# Autodesk Inventor assembly: ASY ДМФ 01 50 Кассета
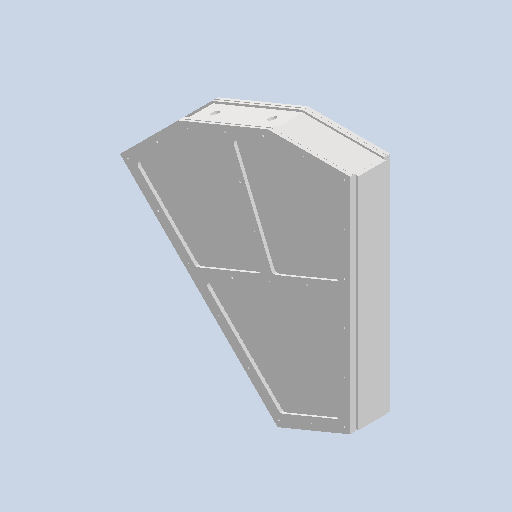
[picture p0: Inventor's stored thumbnail of the model, 512x512]
Saved by Autodesk Inventor 2024.2 (Build 282272000, 272)
## iProperties
Created: 2024-05-05
Part Number: ASY ДМФ 01 50 Кассета
Document SubType Name: Assembly
Designer: pokla
Author: pokla
## Documents named in this file (15)
- C:\Users\pokla\Documents\Inventor\ДФО\ДМФ\DMF-Disk-Micro-Filter-main 16.05.24 12-45\DMF-Disk-Micro-Filter-main\ASY ДМФ 01 50 Кассета.iam
- C:\Users\pokla\Documents\Inventor\ДФО\ДМФ\DMF-Disk-Micro-Filter-main 16.05.24 12-45\DMF-Disk-Micro-Filter-main\ДМФ 01 51 Внешняя рамка.ipt
- ДМС 201 Внешняя рамка.ipt
- C:\Users\pokla\Documents\Inventor\ДФО\ДМФ\DMF-Disk-Micro-Filter-main 16.05.24 12-45\DMF-Disk-Micro-Filter-main\ДМФ 01 52 Верхний лист.ipt
- C:\Users\pokla\Documents\Inventor\ДФО\ДМФ\DMF-Disk-Micro-Filter-main 16.05.24 12-45\DMF-Disk-Micro-Filter-main\ДМФ 01 53 Боковая часть.ipt
- C:\Users\pokla\Documents\Inventor\ДФО\ДМФ\DMF-Disk-Micro-Filter-main 16.05.24 12-45\DMF-Disk-Micro-Filter-main\ДМФ 01 54 Нижний лист.ipt
- C:\Users\pokla\Documents\Inventor\ДФО\ДМФ\DMF-Disk-Micro-Filter-main 16.05.24 12-45\DMF-Disk-Micro-Filter-main\ДМФ 01 55 Усилитель кассеты.ipt
- C:\Users\pokla\Documents\Inventor\ДФО\ДМФ\DMF-Disk-Micro-Filter-main 16.05.24 12-45\DMF-Disk-Micro-Filter-main\ДМФ 01 56 Крепление сетки к кассете.ipt
- ДМС 206 Крепление сетки к кассете.ipt
- C:\Users\pokla\Documents\Inventor\ДФО\ДМФ\DMF-Disk-Micro-Filter-main 16.05.24 12-45\DMF-Disk-Micro-Filter-main\ДМФ 01 57 Сетка кассеты.ipt
- ДМС 207 Сетка кассеты.ipt
- C:\Users\pokla\Documents\Inventor\ДФО\ДМФ\DMF-Disk-Micro-Filter-main 16.05.24 12-45\DMF-Disk-Micro-Filter-main\ДМФ 01 51 Внешние рамки_MIR1.ipt
- C:\Users\pokla\Documents\Inventor\ДФО\ДМФ\DMF-Disk-Micro-Filter-main 16.05.24 12-45\DMF-Disk-Micro-Filter-main\ДМФ 01 56 Крепление сетки к кассете_MIR1.ipt
- C:\Users\pokla\Documents\Inventor\ДФО\ДМФ\DMF-Disk-Micro-Filter-main 16.05.24 12-45\DMF-Disk-Micro-Filter-main\ДМФ 01 57 Сетка кассеты_MIR1.ipt
- C:\Users\pokla\Documents\Inventor\ДФО\ДМФ\DMF-Disk-Micro-Filter-main 16.05.24 12-45\DMF-Disk-Micro-Filter-main\ДМФ 01 58 Фиксатор расстояния кассет.ipt
## Components (12 placed, 11 different names)
1. ДМС 201 Внешняя рамка:1
2. ДМФ 01 52 Верхний лист:1
3. ДМФ 01 53 Боковая часть:1
4. ДМФ 01 54 Нижний лист:1
5. ДМФ 01 55 Усилитель кассеты:1
6. ДМС 206 Крепление сетки к кассете:1
7. ДМС 207 Сетка кассеты:1
8. ДМФ 01 53 Боковая часть:2
9. ДМФ 01 51 Внешние рамки_MIR1:1
10. ДМФ 01 56 Крепление сетки к кассете_MIR1:1
11. ДМФ 01 57 Сетка кассеты_MIR1:1
12. ДМФ 01 58 Фиксатор расстояния кассет:1
## Relationships (12: WeldJoint 8, RevoluteJoint 2, Mate 2)
- [WeldJoint]: ДМС 201 Внешняя рамка:1 ↔ ДМС 207 Сетка кассеты:1
- [WeldJoint]: ДМС 201 Внешняя рамка:1 ↔ ДМФ 01 52 Верхний лист:1
- [RevoluteJoint]: ДМС 201 Внешняя рамка:1 ↔ ДМФ 01 53 Боковая часть:1
- [Mate]: ДМС 201 Внешняя рамка:1 ↔ ДМФ 01 53 Боковая часть:1
- [WeldJoint] (0.5 mm): ДМС 201 Внешняя рамка:1 ↔ ДМС 206 Крепление сетки к кассете:1
- [RevoluteJoint]: ДМС 201 Внешняя рамка:1 ↔ ДМФ 01 53 Боковая часть:2
- [Mate]: ДМС 201 Внешняя рамка:1 ↔ ДМФ 01 53 Боковая часть:2
- [WeldJoint]: ДМС 201 Внешняя рамка:1 ↔ ДМФ 01 54 Нижний лист:1
- [WeldJoint]: ДМС 201 Внешняя рамка:1 ↔ ДМФ 01 55 Усилитель кассеты:1
- [WeldJoint] (0.5 mm): ДМФ 01 51 Внешние рамки_MIR1:1 ↔ ДМФ 01 56 Крепление сетки к кассете_MIR1:1
- [WeldJoint]: ДМФ 01 51 Внешние рамки_MIR1:1 ↔ ДМФ 01 57 Сетка кассеты_MIR1:1
- [WeldJoint]: ДМФ 01 52 Верхний лист:1 ↔ ДМФ 01 58 Фиксатор расстояния кассет:1
## Named parameters: d0_d1 = 0 mm, d1_d3 = 0 mm, d2_d4 = 0 mm, d3_d5 = 90 deg, d4_d6 = 0 mm, d5_d7 = 0.5 mm, d6_d8 = 0 mm, d7_d9 = -90 deg, d8_d10 = 0 mm, d9_d11 = 0 mm
